# Autodesk Inventor assembly: 知能ロボコンばね受け
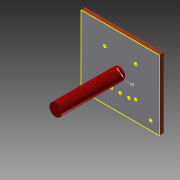
[picture p0: Inventor's stored thumbnail of the model, 180x180]
Saved by Autodesk Inventor 2013 (Build 170138000, 138)
## iProperties
Created: 2014-05-29
Part Number: 知能ロボコンばね受け
Document SubType Name: Assembly
Designer: horumo136
Author: horumo136
## Documents named in this file (3)
- C:\Users\horumo136\Documents\知能ロボコンばね受け.iam
- C:\Users\horumo136\Documents\知能ロボコンばね受け.ipt
- C:\Users\horumo136\Documents\知能ロボコンばね受け受け.ipt
## Components (2 placed, 2 different names)
1. 知能ロボコンばね受け:1 — メイト:1
2. 知能ロボコンばね受け受け:1 — メイト:1
## Relationships (1: Mate 1)
- メイト:1 [Mate]: 知能ロボコンばね受け:1 ↔ 知能ロボコンばね受け受け:1
